# Autodesk Inventor assembly: SAR330 x 2 + regular couplers right offset
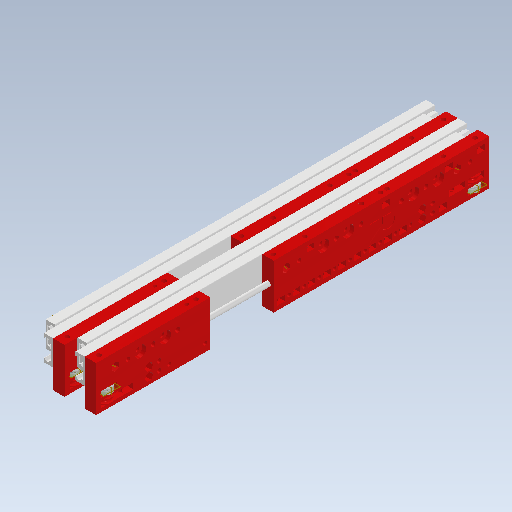
[picture p0: Inventor's stored thumbnail of the model, 512x512]
Saved by Autodesk Inventor 2020 (Build 240168000, 168)
## iProperties
Created: 2019-12-12
Part Number: SAR330 x 2 + regular couplers right offset
Document SubType Name: Assembly
Designer: ball
Author: ball
## Documents named in this file (2)
- D:\FTC8863\2019 Robot\Delivery\Lift Right\SAR330 x 2 + regular couplers right offset.iam
- D:\FTC8863\2019 Robot\Delivery\Lift Right\SAR330 + regular couplers right offset.iam
## Components (2 placed, 1 different names)
1. SAR330 + regular couplers right offset:1 [sub-assembly] — Mate:1, Mate:2, Mate:3
2. SAR330 + regular couplers right offset:2 [sub-assembly] — Mate:1, Mate:2, Mate:3
## Relationships (3: Mate 3)
- Mate:1: SAR330 + regular couplers right offset:1 ↔ SAR330 + regular couplers right offset:2
- Mate:2: SAR330 + regular couplers right offset:1 ↔ SAR330 + regular couplers right offset:2
- Mate:3: SAR330 + regular couplers right offset:1 ↔ SAR330 + regular couplers right offset:2
